# Autodesk Inventor assembly: 12inlift
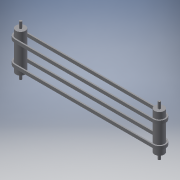
[picture p0: Inventor's stored thumbnail of the model, 180x180]
Saved by Autodesk Inventor 2016 (Build 200138000, 138)
## iProperties
Created: 2016-12-21
Part Number: 12inlift
Document SubType Name: Assembly
Designer: RoboticsUser
Author: RoboticsUser
## Documents named in this file (4)
- C:\Robotics\CAD\2016-17_CAD\12inlift.iam
- C:\Robotics\CAD\2016-17_CAD\LiftLine.ipt
- C:\Robotics\CAD\2016-17_CAD\LiftLineWire.ipt
- C:\Robotics\CAD\2016-17_CAD\4inax.ipt
## Components (6 placed, 3 different names)
1. LiftLine:1 — Flush:2, Mate:2, Flush:5, Mate:5
2. LiftLine:2 — Mate:1, Flush:1, Flush:3, Mate:3, Flush:4, Mate:4
3. LiftLineWire:1 — Mate:1, Flush:1, Flush:2, Mate:2
4. LiftLineWire:2 — Flush:3, Mate:3
5. 4inax:1 — Flush:4, Mate:4
6. 4inax:2 — Flush:5, Mate:5
## Relationships (10: Mate 5, Flush 5)
- Mate:1: LiftLine:2 ↔ LiftLineWire:1
- Flush:1 (-12.7 mm): LiftLine:2 ↔ LiftLineWire:1
- Flush:2 (-12.7 mm): LiftLine:1 ↔ LiftLineWire:1
- Mate:2: LiftLine:1 ↔ LiftLineWire:1
- Flush:3 (12.7 mm): LiftLine:2 ↔ LiftLineWire:2
- Mate:3: LiftLine:2 ↔ LiftLineWire:2
- Flush:4 (-12.7 mm): LiftLine:2 ↔ 4inax:1
- Mate:4: LiftLine:2 ↔ 4inax:1
- Flush:5 (-12.7 mm): LiftLine:1 ↔ 4inax:2
- Mate:5: LiftLine:1 ↔ 4inax:2
